# Autodesk Inventor assembly: BG001_trajan20_21
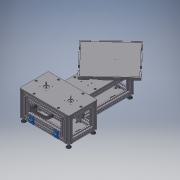
[picture p0: Inventor's stored thumbnail of the model, 180x180]
Saved by Autodesk Inventor 2022.2 (Build 262287000, 287)
## iProperties
Company: HTBLA Kaindorf
RuleStatus: InUse
Created: 2022-08-03
Part Number: BG001_trajan20_21
Project: Zeichenmaschine_v2
Material: Generisch
Description: Gerüst mit Platten
Document SubType Name: Assembly
Designer: trajan20
AfterDocNew0: iProperties-Editor_aufrufen
Author: jan
Keywords: 2021
## Documents named in this file (11)
- C:\Users\jan\Documents\DrawMachine\DrawMachineConstruction\Projekt\Zeichenmaschine_v2\BG001_trajan20_21_Zeichenmaschine_v2_Gerüst mit Platten.iam
- C:\Users\jan\Documents\DrawMachine\DrawMachineConstruction\Projekt\Zeichenmaschine_v2\BT001_trajan20_21_Zeichenmaschine_v2_Platte Stepper Motoren.ipt
- C:\Users\jan\Documents\DrawMachine\DrawMachineConstruction\Projekt\Zeichenmaschine_v2\BT002_trajan20_21_Zeichenmaschine_v2_Platte Getriebemotor.ipt
- C:\Users\jan\Documents\DrawMachine\DrawMachineConstruction\Projekt\Zeichenmaschine_v2\gerüst_v3.iam
- C:\Users\jan\Documents\DrawMachine\DrawMachineConstruction\Projekt\Zeichenmaschine_v2\importierte bauteile\Steppermotor.ipt
- C:\Users\jan\Documents\DrawMachine\DrawMachineConstruction\Projekt\Zeichenmaschine_v2\importierte bauteile\Getriebemotor.ipt
- C:\Users\jan\Documents\DrawMachine\DrawMachineConstruction\Projekt\Zeichenmaschine_v2\BT005_trajan20_21_Zeichenmaschine_v2_getriebemotor platte unten.ipt
- C:\Users\jan\Documents\DrawMachine\DrawMachineConstruction\Projekt\Zeichenmaschine_v2\BT004_trajan20_21_Zeichenmaschine_v2_Hauptplatte unten.ipt
- C:\Users\jan\Documents\DrawMachine\DrawMachineConstruction\Projekt\Zeichenmaschine_v2\BT003_trajan20_21_Zeichenmaschine_v2_zwischenteil platte gm.ipt
- C:\Users\jan\Documents\DrawMachine\DrawMachineConstruction\Projekt\Zeichenmaschine_v2\BT001_trajan20_21_Zeichenmaschine_v2_zentrierhülse platte.ipt
- C:\Users\jan\Documents\DrawMachine\DrawMachineConstruction\Projekt\Zeichenmaschine_v2\BT002_trajan20_21_Zeichenmaschine_v2_papierplatte.ipt
## Components (11 placed, 10 different names)
1. BT001_trajan20_21_Zeichenmaschine_v2_Platte Stepper Motoren:1 — Fluchtend:3, Fluchtend:4, Passend:2, Passend:3, Passend:4, Passend:5, Passend:6
2. BT002_trajan20_21_Zeichenmaschine_v2_Platte Getriebemotor:1 — Fluchtend:1, Fluchtend:2, Passend:1, Passend:7, Passend:8, Passend:16
3. gerüst_v3:1 [sub-assembly] — Fluchtend:1, Fluchtend:2, Passend:1, Fluchtend:3, Fluchtend:4, Passend:2, Winkel:1, Winkel:2, Winkel:3, Passend:9, Passend:10, Passend:11, Passend:12, Passend:13, Passend:14
4. Steppermotor:1 — Passend:5, Passend:6, Winkel:2
5. Steppermotor:2 — Passend:3, Winkel:1, Passend:4
6. Getriebemotor:1 — Passend:7, Winkel:3, Passend:8, Passend:15
7. BT005_trajan20_21_Zeichenmaschine_v2_getriebemotor platte unten:1 — Passend:9, Passend:10, Passend:11
8. BT004_trajan20_21_Zeichenmaschine_v2_Hauptplatte unten:1 — Passend:12, Passend:13, Passend:14
9. BT003_trajan20_21_Zeichenmaschine_v2_zwischenteil platte gm:1 — Passend:15, Passend:16, Passend:17, Passend:18, Passend:20, Passend:21
10. BT001_trajan20_21_Zeichenmaschine_v2_zentrierhülse platte:1 — Passend:17, Passend:18, Passend:19
11. BT002_trajan20_21_Zeichenmaschine_v2_papierplatte:1 — Passend:19, Passend:20, Passend:21
## Relationships (28: Mate 21, Flush 4, Angle 3)
- Fluchtend:1 [Flush]: BT002_trajan20_21_Zeichenmaschine_v2_Platte Getriebemotor:1 ↔ gerüst_v3:1
- Fluchtend:2 [Flush]: BT002_trajan20_21_Zeichenmaschine_v2_Platte Getriebemotor:1 ↔ gerüst_v3:1
- Passend:1 [Mate]: BT002_trajan20_21_Zeichenmaschine_v2_Platte Getriebemotor:1 ↔ gerüst_v3:1
- Fluchtend:3 [Flush]: BT001_trajan20_21_Zeichenmaschine_v2_Platte Stepper Motoren:1 ↔ gerüst_v3:1
- Fluchtend:4 [Flush]: BT001_trajan20_21_Zeichenmaschine_v2_Platte Stepper Motoren:1 ↔ gerüst_v3:1
- Passend:2 [Mate]: BT001_trajan20_21_Zeichenmaschine_v2_Platte Stepper Motoren:1 ↔ gerüst_v3:1
- Passend:3 [Mate]: BT001_trajan20_21_Zeichenmaschine_v2_Platte Stepper Motoren:1 ↔ Steppermotor:2
- Winkel:1 [Angle] (0 deg): gerüst_v3:1 ↔ Steppermotor:2
- Passend:4 [Mate]: BT001_trajan20_21_Zeichenmaschine_v2_Platte Stepper Motoren:1 ↔ Steppermotor:2
- Passend:5 [Mate]: BT001_trajan20_21_Zeichenmaschine_v2_Platte Stepper Motoren:1 ↔ Steppermotor:1
- Passend:6 [Mate]: BT001_trajan20_21_Zeichenmaschine_v2_Platte Stepper Motoren:1 ↔ Steppermotor:1
- Winkel:2 [Angle] (0 deg): gerüst_v3:1 ↔ Steppermotor:1
- Passend:7 [Mate]: BT002_trajan20_21_Zeichenmaschine_v2_Platte Getriebemotor:1 ↔ Getriebemotor:1
- Winkel:3 [Angle] (0 deg): gerüst_v3:1 ↔ Getriebemotor:1
- Passend:8 [Mate]: BT002_trajan20_21_Zeichenmaschine_v2_Platte Getriebemotor:1 ↔ Getriebemotor:1
- Passend:9 [Mate]: gerüst_v3:1 ↔ BT005_trajan20_21_Zeichenmaschine_v2_getriebemotor platte unten:1
- Passend:10 [Mate]: gerüst_v3:1 ↔ BT005_trajan20_21_Zeichenmaschine_v2_getriebemotor platte unten:1
- Passend:11 [Mate]: gerüst_v3:1 ↔ BT005_trajan20_21_Zeichenmaschine_v2_getriebemotor platte unten:1
- Passend:12 [Mate]: gerüst_v3:1 ↔ BT004_trajan20_21_Zeichenmaschine_v2_Hauptplatte unten:1
- Passend:13 [Mate]: gerüst_v3:1 ↔ BT004_trajan20_21_Zeichenmaschine_v2_Hauptplatte unten:1
- Passend:14 [Mate]: gerüst_v3:1 ↔ BT004_trajan20_21_Zeichenmaschine_v2_Hauptplatte unten:1
- Passend:15 [Mate]: Getriebemotor:1 ↔ BT003_trajan20_21_Zeichenmaschine_v2_zwischenteil platte gm:1
- Passend:16 [Mate]: BT002_trajan20_21_Zeichenmaschine_v2_Platte Getriebemotor:1 ↔ BT003_trajan20_21_Zeichenmaschine_v2_zwischenteil platte gm:1
- Passend:17 [Mate]: BT003_trajan20_21_Zeichenmaschine_v2_zwischenteil platte gm:1 ↔ BT001_trajan20_21_Zeichenmaschine_v2_zentrierhülse platte:1
- Passend:18 [Mate]: BT003_trajan20_21_Zeichenmaschine_v2_zwischenteil platte gm:1 ↔ BT001_trajan20_21_Zeichenmaschine_v2_zentrierhülse platte:1
- Passend:19 [Mate]: BT001_trajan20_21_Zeichenmaschine_v2_zentrierhülse platte:1 ↔ BT002_trajan20_21_Zeichenmaschine_v2_papierplatte:1
- Passend:20 [Mate]: BT003_trajan20_21_Zeichenmaschine_v2_zwischenteil platte gm:1 ↔ BT002_trajan20_21_Zeichenmaschine_v2_papierplatte:1
- Passend:21 [Mate]: BT003_trajan20_21_Zeichenmaschine_v2_zwischenteil platte gm:1 ↔ BT002_trajan20_21_Zeichenmaschine_v2_papierplatte:1
